# Autodesk Inventor assembly: Motor_Panel
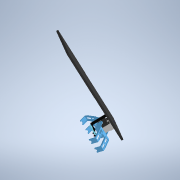
[picture p0: Inventor's stored thumbnail of the model, 180x180]
Saved by Autodesk Inventor 2020 (Build 240168000, 168)
## iProperties
Created: 2019-09-17
Part Number: Motor_Panel
Document SubType Name: Assembly
Designer: Knowblesse
Author: Knowblesse
## Documents named in this file (11)
- C:\VCF\Lobster\Apparatus\Visual\Motor_Panel.iam
- C:\VCF\Lobster\Apparatus\Visual\Motor.ipt
- C:\VCF\Lobster\Apparatus\Visual\Motor_disk.ipt
- C:\VCF\Lobster\Apparatus\MotorBracket.ipt
- C:\VCF\Lobster\Apparatus\Visual\Board.ipt
- C:\VCF\Lobster\Apparatus\servo_bracket_claw_left_v5-JY.ipt
- C:\VCF\Lobster\Apparatus\servo_bracket_claw_right_v5-JY.ipt
- C:\VCF\Lobster\Apparatus\LickModuleMount_Training.ipt
- C:\VCF\Lobster\Apparatus\LickSensorMount.ipt
- C:\VCF\Lobster\Apparatus\Visual\LickSensor.ipt
- C:\VCF\Lobster\Apparatus\Visual\LickLight.ipt
## Components (13 placed, 10 different names)
1. Motor:1 — 회전:1, 강체:1
2. Motor:2 — 회전:2, 강체:2
3. Motor_disk:1 — 회전:2, 회전:4
4. Motor_disk:2 — 회전:1, 회전:3
5. MotorBracket:1 — 강체:1, 강체:2, 강체:3
6. Board:1 — 강체:3, 강체:5
7. servo_bracket_claw_left_v5-JY:1 — 회전:4
8. servo_bracket_claw_right_v5-JY:1 — 회전:3
9. LickModuleMount_Training:1 — 강체:4, 강체:5
10. LickSensorMount:1 — 강체:4, 강체:6, 강체:7
11. LickSensor:1 — 강체:7, 강체:8
12. LickSensor:2 — 강체:6
13. LickLight:1 — 강체:8
## Relationships (12: WeldJoint 8, RevoluteJoint 4)
- 회전:1 [RevoluteJoint]: Motor:1 ↔ Motor_disk:2
- 회전:2 [RevoluteJoint]: Motor:2 ↔ Motor_disk:1
- 강체:1 [WeldJoint]: Motor:1 ↔ MotorBracket:1
- 강체:2 [WeldJoint]: Motor:2 ↔ MotorBracket:1
- 강체:3 [WeldJoint]: MotorBracket:1 ↔ Board:1
- 회전:3 [RevoluteJoint]: Motor_disk:2 ↔ servo_bracket_claw_right_v5-JY:1
- 회전:4 [RevoluteJoint]: Motor_disk:1 ↔ servo_bracket_claw_left_v5-JY:1
- 강체:4 [WeldJoint]: LickModuleMount_Training:1 ↔ LickSensorMount:1
- 강체:5 [WeldJoint]: Board:1 ↔ LickModuleMount_Training:1
- 강체:6 [WeldJoint]: LickSensorMount:1 ↔ LickSensor:2
- 강체:7 [WeldJoint]: LickSensorMount:1 ↔ LickSensor:1
- 강체:8 [WeldJoint]: LickSensor:1 ↔ LickLight:1
